# Autodesk Inventor assembly: A2017_T2_04
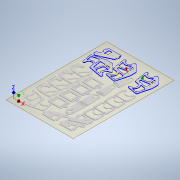
[picture p0: Inventor's stored thumbnail of the model, 180x180]
Saved by Autodesk Inventor 2020 (Build 240168000, 168)
## iProperties
Created: 2021-08-27
Part Number: A2017_T2_04
Document SubType Name: Assembly
Designer: Masato
Author: Masato
## Documents named in this file (8)
- C:\Users\L20C1118 森　圭汰\Documents\220111_openplatform\OpenPlatform_ver3_0\cam\A2017_T2_04.iam
- C:\Users\L20C1118 森　圭汰\Documents\220111_openplatform\OpenPlatform_ver3_0\cam\Disposable_Board.ipt
- C:\Users\L20C1118 森　圭汰\Documents\220111_openplatform\OpenPlatform_ver3_0\LowerBody\Ankle\Ankle_side_frame.ipt
- C:\Users\L20C1118 森　圭汰\Documents\220111_openplatform\OpenPlatform_ver3_0\LowerBody\Ankle\Ankle_back_frame.ipt
- C:\Users\L20C1118 森　圭汰\Documents\220111_openplatform\OpenPlatform_ver3_0\LowerBody\Foot\Foot_back_frame.ipt
- C:\Users\L20C1118 森　圭汰\Documents\220111_openplatform\OpenPlatform_ver3_0\LowerBody\Foot\Foot_front_frame.ipt
- C:\Users\L20C1118 森　圭汰\Documents\220111_openplatform\OpenPlatform_ver3_0\LowerBody\Leg_joit\Leg_joint_pitch_frame.ipt
- C:\Users\L20C1118 森　圭汰\Documents\220111_openplatform\OpenPlatform_ver3_0\LowerBody\Knee\Knee_side_frame.ipt
## Components (21 placed, 7 different names)
1. Disposable_Board:1 — メイト:2, メイト:1, フラッシュ:1, フラッシュ:2, フラッシュ:7, フラッシュ:8, 正接:2, 正接:3, フラッシュ:10, 正接:4, 正接:5, フラッシュ:11, フラッシュ:13, フラッシュ:17, 正接:10
2. Ankle_side_frame:1 — メイト:20, フラッシュ:3, メイト:24, フラッシュ:7, 正接:1, メイト:30
3. Ankle_side_frame:2 — メイト:21, フラッシュ:3, フラッシュ:4, メイト:24, メイト:25
4. Ankle_side_frame:3 — メイト:23, フラッシュ:5, メイト:26, フラッシュ:9
5. Ankle_side_frame:4 — メイト:22, フラッシュ:4, フラッシュ:5, メイト:25, メイト:26
6. Ankle_back_frame:1 — メイト:14, フラッシュ:21, メイト:36
7. Ankle_back_frame:2 — メイト:12, フラッシュ:19, フラッシュ:20, メイト:34, メイト:35
8. Ankle_back_frame:3 — メイト:13, フラッシュ:20, フラッシュ:21, メイト:35, メイト:36
9. Ankle_back_frame:4 — メイト:15, フラッシュ:18, フラッシュ:19, メイト:33, メイト:34
10. Foot_back_frame:1 — メイト:16, フラッシュ:15, メイト:31, 正接:9, フラッシュ:16
11. Foot_back_frame:2 — メイト:17, メイト:30, フラッシュ:15, メイト:31, 正接:8
12. Foot_front_frame:1 — メイト:18, 正接:9, フラッシュ:16, 正接:11
13. Foot_front_frame:2 — メイト:19, 正接:11, メイト:32
14. Leg_joint_pitch_frame:1 — メイト:11, フラッシュ:10, 正接:4
15. Leg_joint_pitch_frame:2 — メイト:8, メイト:29, フラッシュ:12, 正接:6, フラッシュ:14
16. Leg_joint_pitch_frame:3 — メイト:10, フラッシュ:14, 正接:7, 正接:8
17. Leg_joint_pitch_frame:4 — メイト:9, メイト:29, フラッシュ:13, 正接:6, フラッシュ:18, メイト:33
18. Knee_side_frame:1 — メイト:28, フラッシュ:9, 正接:3
19. Knee_side_frame:2 — メイト:6, 正接:5, フラッシュ:11, メイト:32
20. Knee_side_frame:3 — メイト:7, フラッシュ:17, 正接:10
21. Knee_side_frame:4 — メイト:27, フラッシュ:8, 正接:1, 正接:2, フラッシュ:12, 正接:7
## Relationships (64: Mate 33, Flush 20, Tangent 11)
- メイト:2 [Mate]: Disposable_Board:1
- メイト:1 [Mate]: Disposable_Board:1
- フラッシュ:1 [Flush]: Disposable_Board:1
- フラッシュ:2 [Flush]: Disposable_Board:1
- メイト:6 [Mate]: Knee_side_frame:2
- メイト:7 [Mate]: Knee_side_frame:3
- メイト:8 [Mate]: Leg_joint_pitch_frame:2
- メイト:9 [Mate]: Leg_joint_pitch_frame:4
- メイト:10 [Mate]: Leg_joint_pitch_frame:3
- メイト:11 [Mate]: Leg_joint_pitch_frame:1
- メイト:12 [Mate]: Ankle_back_frame:2
- メイト:13 [Mate]: Ankle_back_frame:3
- メイト:14 [Mate]: Ankle_back_frame:1
- メイト:15 [Mate]: Ankle_back_frame:4
- メイト:16 [Mate]: Foot_back_frame:1
- メイト:17 [Mate]: Foot_back_frame:2
- メイト:18 [Mate]: Foot_front_frame:1
- メイト:19 [Mate]: Foot_front_frame:2
- メイト:20 [Mate]: Ankle_side_frame:1
- メイト:21 [Mate]: Ankle_side_frame:2
- メイト:22 [Mate]: Ankle_side_frame:4
- メイト:23 [Mate]: Ankle_side_frame:3
- フラッシュ:3 [Flush]: Ankle_side_frame:1 ↔ Ankle_side_frame:2
- フラッシュ:4 [Flush]: Ankle_side_frame:2 ↔ Ankle_side_frame:4
- フラッシュ:5 [Flush]: Ankle_side_frame:3 ↔ Ankle_side_frame:4
- メイト:24 [Mate] (5 mm): Ankle_side_frame:1 ↔ Ankle_side_frame:2
- メイト:25 [Mate] (5 mm): Ankle_side_frame:2 ↔ Ankle_side_frame:4
- メイト:26 [Mate] (5 mm): Ankle_side_frame:3 ↔ Ankle_side_frame:4
- メイト:27 [Mate]: Knee_side_frame:4
- フラッシュ:7 [Flush] (3 mm): Disposable_Board:1 ↔ Ankle_side_frame:1
- フラッシュ:8 [Flush] (3 mm): Disposable_Board:1 ↔ Knee_side_frame:4
- 正接:1 [Tangent] (3 mm): Ankle_side_frame:1 ↔ Knee_side_frame:4
- 正接:2 [Tangent] (3 mm): Disposable_Board:1 ↔ Knee_side_frame:4
- メイト:28 [Mate]: Knee_side_frame:1
- フラッシュ:9 [Flush] (-70 mm): Ankle_side_frame:3 ↔ Knee_side_frame:1
- 正接:3 [Tangent] (3 mm): Disposable_Board:1 ↔ Knee_side_frame:1
- フラッシュ:10 [Flush] (3 mm): Disposable_Board:1 ↔ Leg_joint_pitch_frame:1
- 正接:4 [Tangent] (3 mm): Disposable_Board:1 ↔ Leg_joint_pitch_frame:1
- 正接:5 [Tangent] (3 mm): Disposable_Board:1 ↔ Knee_side_frame:2
- フラッシュ:11 [Flush] (75 mm): Disposable_Board:1 ↔ Knee_side_frame:2
- メイト:29 [Mate] (3 mm): Leg_joint_pitch_frame:2 ↔ Leg_joint_pitch_frame:4
- フラッシュ:12 [Flush]: Leg_joint_pitch_frame:2 ↔ Knee_side_frame:4
- フラッシュ:13 [Flush] (-3 mm): Disposable_Board:1 ↔ Leg_joint_pitch_frame:4
- 正接:6 [Tangent]: Leg_joint_pitch_frame:2 ↔ Leg_joint_pitch_frame:4
- フラッシュ:14 [Flush]: Leg_joint_pitch_frame:2 ↔ Leg_joint_pitch_frame:3
- 正接:7 [Tangent] (3 mm): Leg_joint_pitch_frame:3 ↔ Knee_side_frame:4
- メイト:30 [Mate] (4 mm): Ankle_side_frame:1 ↔ Foot_back_frame:2
- フラッシュ:15 [Flush]: Foot_back_frame:1 ↔ Foot_back_frame:2
- メイト:31 [Mate] (3 mm): Foot_back_frame:1 ↔ Foot_back_frame:2
- 正接:8 [Tangent] (3 mm): Foot_back_frame:2 ↔ Leg_joint_pitch_frame:3
- 正接:9 [Tangent] (3 mm): Foot_back_frame:1 ↔ Foot_front_frame:1
- フラッシュ:16 [Flush]: Foot_back_frame:1 ↔ Foot_front_frame:1
- フラッシュ:17 [Flush] (3 mm): Disposable_Board:1 ↔ Knee_side_frame:3
- 正接:10 [Tangent] (3 mm): Disposable_Board:1 ↔ Knee_side_frame:3
- 正接:11 [Tangent] (3 mm): Foot_front_frame:1 ↔ Foot_front_frame:2
- メイト:32 [Mate] (3 mm): Foot_front_frame:2 ↔ Knee_side_frame:2
- フラッシュ:18 [Flush]: Ankle_back_frame:4 ↔ Leg_joint_pitch_frame:4
- フラッシュ:19 [Flush]: Ankle_back_frame:2 ↔ Ankle_back_frame:4
- フラッシュ:20 [Flush]: Ankle_back_frame:2 ↔ Ankle_back_frame:3
- フラッシュ:21 [Flush]: Ankle_back_frame:1 ↔ Ankle_back_frame:3
- メイト:33 [Mate] (3 mm): Ankle_back_frame:4 ↔ Leg_joint_pitch_frame:4
- メイト:34 [Mate] (3 mm): Ankle_back_frame:2 ↔ Ankle_back_frame:4
- メイト:35 [Mate] (3 mm): Ankle_back_frame:2 ↔ Ankle_back_frame:3
- メイト:36 [Mate] (3 mm): Ankle_back_frame:1 ↔ Ankle_back_frame:3
